# Autodesk Inventor assembly: Intake Assembly
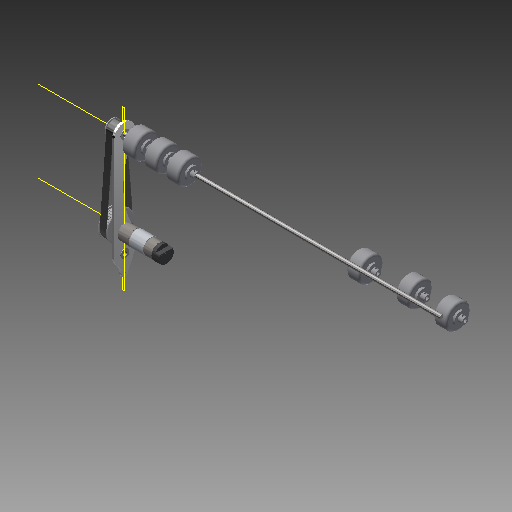
[picture p0: Inventor's stored thumbnail of the model, 512x512]
Saved by Autodesk Inventor 2019.4 (Build 234330000, 330)
## iProperties
Created: 2020-01-05
Part Number: Intake Assembly
Document SubType Name: Assembly
Designer: admin
Author: admin
## Documents named in this file (7)
- C:\Users\Mark\Desktop\7738 Helion Engineering\7738-2020\Intake Mechanism\Intake Assembly.iam
- C:\Users\Mark\Desktop\7738 Helion Engineering\7738-2020\Intake Mechanism\Main Axle.ipt
- C:\Users\Mark\Desktop\7738 Helion Engineering\7738-2020\Intake Mechanism\Intake Arm Left.ipt
- C:\Users\Mark\Desktop\7738 Helion Engineering\7738-2020\CAD\Gearbox\F6800.ipt
- C:\Users\Mark\Desktop\7738 Helion Engineering\7738-2020\Intake Mechanism\Neverest\am-3103 NeveRest 60.ipt
- C:\Users\Mark\Desktop\7738 Helion Engineering\7738-2020\Intake Mechanism\Intake Assembly\Design Accelerator\Synchronous Belts Transmission1.iam
- C:\Users\Mark\Desktop\7738 Helion Engineering\7738-2020\Intake Mechanism\Mecanum Wheel.ipt
## Components (12 placed, 6 different names)
1. Main Axle:1 — Mate:9, Flush:2, Mate:10, Mate:11, Mate:12
2. Intake Arm Left:1 — Mate:1, Mate:2, Mate:3, Mate:4, Mate:6, Mate:7, Flush:1, Mate:8
3. F6800:1 — Mate:1, Mate:4, Mate:9
4. F6800:2 — Mate:2, Mate:3
5. am-3103 NeveRest 60:1 — Mate:6, Mate:7, Mate:8
6. Synchronous Belts Transmission:1 [sub-assembly] — Flush:2
7. Mecanum Wheel:1 — Mate:10, Mate:13
8. Mecanum Wheel:2 — Mate:11, Mate:13, Mate:14
9. Mecanum Wheel:3 — Mate:12, Mate:14
10. Mecanum Wheel:4
11. Mecanum Wheel:5
12. Mecanum Wheel:6
## Relationships (15: Mate 13, Flush 2)
- Mate:1: Intake Arm Left:1 ↔ F6800:1
- Mate:2: Intake Arm Left:1 ↔ F6800:2
- Mate:3 (0.2 mm): Intake Arm Left:1 ↔ F6800:2
- Mate:4 (0.2 mm): Intake Arm Left:1 ↔ F6800:1
- Mate:6: Intake Arm Left:1 ↔ am-3103 NeveRest 60:1
- Mate:7 (0.2 mm): Intake Arm Left:1 ↔ am-3103 NeveRest 60:1
- Flush:1 (-25 mm): Intake Arm Left:1
- Mate:8: Intake Arm Left:1 ↔ am-3103 NeveRest 60:1
- Mate:9: Main Axle:1 ↔ F6800:1
- Flush:2: Main Axle:1 ↔ Synchronous Belts Transmission:1
- Mate:10: Main Axle:1 ↔ Mecanum Wheel:1
- Mate:11: Main Axle:1 ↔ Mecanum Wheel:2
- Mate:12: Main Axle:1 ↔ Mecanum Wheel:3
- Mate:13 (5 mm): Mecanum Wheel:1 ↔ Mecanum Wheel:2
- Mate:14 (5 mm): Mecanum Wheel:2 ↔ Mecanum Wheel:3
